# Autodesk Inventor assembly: wheel assembly
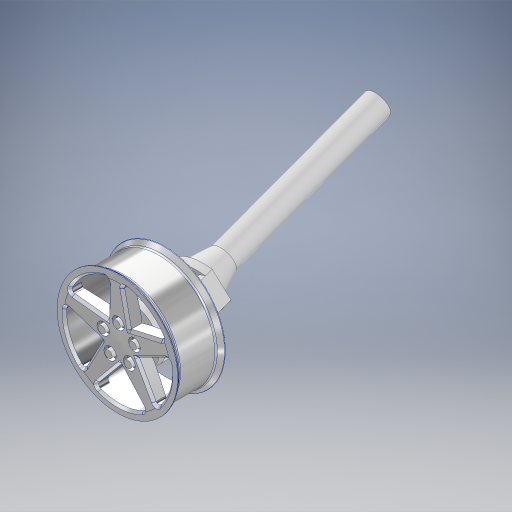
[picture p0: Inventor's stored thumbnail of the model, 512x512]
Saved by Autodesk Inventor 2024 (Build 280153000, 153)
## iProperties
Created: 2024-04-03
Part Number: wheel assembly
Document SubType Name: Assembly
Designer: Alex
Author: Alex
## Documents named in this file (5)
- C:\Shared\alex-bartella-schoolwork\4z03\final\wheel assembly.iam
- C:\Shared\alex-bartella-schoolwork\4z03\final\wheel hub.ipt
- C:\Shared\alex-bartella-schoolwork\4z03\final\wheel.ipt
- C:\Shared\alex-bartella-schoolwork\4z03\final\u joint.ipt
- C:\Shared\alex-bartella-schoolwork\4z03\final\driveshaft.ipt
## Components (4 placed, 4 different names)
1. wheel hub:1 — Mate:1, Mate:2, Mate:3, Mate:5, Flush:2
2. wheel:1 — Mate:1, Mate:2, Mate:3, Mate:4, Flush:1
3. u joint:1 — Mate:5, Flush:2, Mate:6, Flush:3
4. driveshaft:1 — Mate:6, Flush:3
## Relationships (9: Mate 6, Flush 3)
- Mate:1: wheel hub:1 ↔ wheel:1
- Mate:2: wheel hub:1 ↔ wheel:1
- Mate:3: wheel hub:1 ↔ wheel:1
- Mate:4: wheel:1
- Flush:1: wheel:1
- Mate:5: wheel hub:1 ↔ u joint:1
- Flush:2 (-2 mm): wheel hub:1 ↔ u joint:1
- Mate:6: u joint:1 ↔ driveshaft:1
- Flush:3 (2 mm): u joint:1 ↔ driveshaft:1
